# Autodesk Inventor assembly: ASSEMBLY_Bucket_tooth
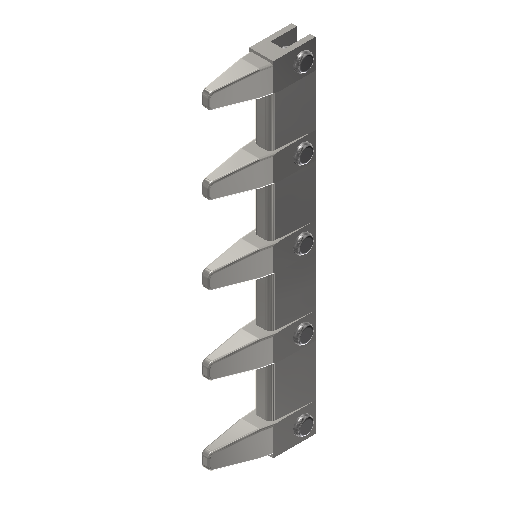
[picture p0: Inventor's stored thumbnail of the model, 512x512]
Saved by Autodesk Inventor 2025 (Build 290162010, 162A)
## iProperties
Created: 2018-09-17
Part Number: ASSEMBLY_Bucket_tooth
Document SubType Name: Assembly
Designer: Andrzej
Mass: 16.4853 g
Surface Area: 32.2774 cm^2
Volume: 2.06067 cm^3
Density: 8 g/cm^3
Author: Andrzej
## Documents named in this file (3)
- D:\_ANDRZEJ_LACZEWSKI\_OTHER\MECH - My entry for the NASA Lunar Sampling System Design Challenge\MCAD\1_REV1\ASSEMBLY_MAIN_REVA\ASSEMBLY_Bucket_tooth.iam
- D:\_ANDRZEJ_LACZEWSKI\_OTHER\MECH - My entry for the NASA Lunar Sampling System Design Challenge\MCAD\1_REV1\ASSEMBLY_MAIN_REVA\CNCT_STEEL_Bucket_tooth_mounting_pin.ipt
- D:\_ANDRZEJ_LACZEWSKI\_OTHER\MECH - My entry for the NASA Lunar Sampling System Design Challenge\MCAD\1_REV1\ASSEMBLY_MAIN_REVA\CNCM_TITANIUM_Bucket_Tooth.ipt
## Components (6 placed, 2 different names)
1. CNCT_STEEL_Bucket_tooth_mounting_pin:1 — Mate:2, Mate:8
2. CNCT_STEEL_Bucket_tooth_mounting_pin:2 — Mate:1, Mate:6
3. CNCT_STEEL_Bucket_tooth_mounting_pin:3 — Mate:3, Mate:9
4. CNCT_STEEL_Bucket_tooth_mounting_pin:4 — Mate:4, Mate:10
5. CNCT_STEEL_Bucket_tooth_mounting_pin:5 — Mate:5, Mate:7
6. CNCM_TITANIUM_Bucket_Tooth:1 — Mate:1, Mate:2, Mate:3, Mate:4, Mate:5, Mate:6, Mate:7, Mate:8, Mate:9, Mate:10
## Relationships (10: Mate 10)
- Mate:1: CNCT_STEEL_Bucket_tooth_mounting_pin:2 ↔ CNCM_TITANIUM_Bucket_Tooth:1
- Mate:2: CNCT_STEEL_Bucket_tooth_mounting_pin:1 ↔ CNCM_TITANIUM_Bucket_Tooth:1
- Mate:3: CNCT_STEEL_Bucket_tooth_mounting_pin:3 ↔ CNCM_TITANIUM_Bucket_Tooth:1
- Mate:4: CNCT_STEEL_Bucket_tooth_mounting_pin:4 ↔ CNCM_TITANIUM_Bucket_Tooth:1
- Mate:5: CNCT_STEEL_Bucket_tooth_mounting_pin:5 ↔ CNCM_TITANIUM_Bucket_Tooth:1
- Mate:6: CNCT_STEEL_Bucket_tooth_mounting_pin:2 ↔ CNCM_TITANIUM_Bucket_Tooth:1
- Mate:7: CNCT_STEEL_Bucket_tooth_mounting_pin:5 ↔ CNCM_TITANIUM_Bucket_Tooth:1
- Mate:8: CNCT_STEEL_Bucket_tooth_mounting_pin:1 ↔ CNCM_TITANIUM_Bucket_Tooth:1
- Mate:9: CNCT_STEEL_Bucket_tooth_mounting_pin:3 ↔ CNCM_TITANIUM_Bucket_Tooth:1
- Mate:10: CNCT_STEEL_Bucket_tooth_mounting_pin:4 ↔ CNCM_TITANIUM_Bucket_Tooth:1
